# Autodesk Inventor assembly: Laufkatze_Baugruppe_neu
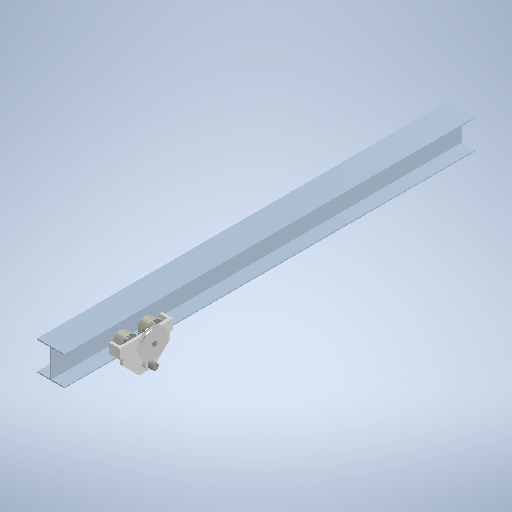
[picture p0: Inventor's stored thumbnail of the model, 512x512]
Saved by Autodesk Inventor 2025.2 (Build 292293000, 293)
## iProperties
Created: 2025-02-05
Part Number: Laufkatze_Baugruppe_neu
Document SubType Name: Assembly
Designer: akoca
Author: akoca
## Documents named in this file (16)
- C:\Users\akoca\Documents\MCI\Semester_3\AMEII\Projekt\Laufkatze\Baugruppen\Laufkatze_Baugruppe_neu.iam
- C:\Users\akoca\Documents\MCI\Semester_3\AMEII\Projekt\Laufkatze\Einzelbauteile\Stahlträger.ipt
- C:\Users\akoca\Documents\MCI\Semester_3\AMEII\Projekt\Laufkatze\Einzelbauteile\Zahnrad_für_Kettenzug.ipt
- C:\Users\akoca\Documents\MCI\Semester_3\AMEII\Projekt\Laufkatze\Einzelbauteile\Zahnrad_bei_Laufrad.ipt
- C:\Users\akoca\Documents\MCI\Semester_3\AMEII\Projekt\Laufkatze\Einzelbauteile\Laufrad.ipt
- C:\Users\akoca\Documents\MCI\Semester_3\AMEII\Projekt\Laufkatze\Einzelbauteile\Welle_für_Kettenzug.ipt
- C:\Users\akoca\Documents\MCI\Semester_3\AMEII\Projekt\Laufkatze\Einzelbauteile\Führungsplatte_rechts.ipt
- C:\Users\akoca\Documents\MCI\Semester_3\AMEII\Projekt\Laufkatze\Baugruppen\Laufkatze_Baugruppe\Konstruktions-Assistent\Lager4.iam
- C:\Users\akoca\Documents\MCI\Semester_3\AMEII\Projekt\Laufkatze\Einzelbauteile\Zugscheibe_für_Kette.ipt
- C:\Users\akoca\Documents\MCI\Semester_3\AMEII\Projekt\Laufkatze\Einzelbauteile\Führungsplatte_links.ipt
- C:\Users\akoca\Documents\MCI\Semester_3\AMEII\Projekt\Laufkatze\Einzelbauteile\Schraubbolzen.ipt
- C:\Users\akoca\Documents\MCI\Semester_3\AMEII\Projekt\Laufkatze\Baugruppen\Laufkatze_Baugruppe\Konstruktions-Assistent\Lager1.iam
- C:\Users\akoca\Documents\MCI\Semester_3\AMEII\Projekt\Laufkatze\Normteile\de-DE\DIN EN ISO 7093-2\DIN EN ISO 7093-2 - 14.ipt
- C:\Users\akoca\Documents\MCI\Semester_3\AMEII\Projekt\Laufkatze\Normteile\de-DE\ISO 8676(1)\ISO 8676 - M12 x 1,25 x 30DIN EN.ipt
- C:\Users\akoca\Documents\MCI\Semester_3\AMEII\Projekt\Laufkatze\Normteile\de-DE\DIN EN ISO 7093-2\DIN EN ISO 7093-2 - 12.ipt
- C:\Users\akoca\Documents\MCI\Semester_3\AMEII\Projekt\Laufkatze\Skelett_Laufkatze.ipt
## Components (29 placed, 13 different names)
1. DIN EN 28676 M12 x 1,25 x 30:6 — Drehbar:21
2. DIN EN ISO 7093-2 12:1 — Starr:11, Drehbar:21
3. DIN EN 28676 M12 x 1,25 x 30:5 — Starr:10
4. DIN EN 28676 M12 x 1,25 x 30:4 — Drehbar:19
5. DIN EN ISO 7093-2 14:4 — Starr:8, Drehbar:19
6. DIN EN 28676 M12 x 1,25 x 30:3 — Drehbar:20
7. DIN EN ISO 7093-2 14:3 — Starr:9, Drehbar:20
8. DIN EN 28676 M12 x 1,25 x 30:2 — Drehbar:18
9. DIN EN ISO 7093-2 14:2 — Starr:6, Drehbar:18
10. DIN EN ISO 7093-2 14:1 — Starr:7, Starr:10
11. Lager:6 [sub-assembly] — Drehbar:17
12. Lager:5 [sub-assembly] — Drehbar:16
13. Lager:4 [sub-assembly] — Drehbar:15
14. Lager:3 [sub-assembly] — Drehbar:14
15. Lager:2 [sub-assembly] — Starr:5
16. Lager:1 [sub-assembly] — Starr:4
17. Schraubbolzen:1 — Passend:7, Passend:8, Fluchtend:3
18. Laufrad:4 — Drehbar:12, Tangential:6, Drehbar:14
19. Laufrad:3 — Drehbar:13, Tangential:5, Passend:9, Drehbar:15
20. Führungsplatte_links:1 — Drehbar:12, Drehbar:13, Passend:8, Starr:6, Starr:7
21. Zugscheibe_für_Kette:1 — Drehbar:9, Drehung:3
22. Führungsplatte_rechts:1 — Drehbar:8, Drehbar:7, Passend:7, Starr:8, Starr:9, Fluchtend:4
23. Welle_für_Kettenzug:1 — Starr:4, Starr:5, Zahnrad-Bewegung, Drehbar:9, Starr:11
24. Laufrad:2 — Passend:2, Tangential:3, Starr:2, Passend:6, Drehbar:16
25. Laufrad:1 — Passend:4, Tangential:4, Starr:1, Passend:5, Drehung/Translation:1, Drehbar:17
26. Zahnrad_bei_Laufrad:2 — Fluchtend:2, Tangential:1, Passend:4, Starr:1, Drehbar:8, Drehung:2
27. Zahnrad_bei_Laufrad:1 — Fluchtend:1, Tangential:2, Passend:2, Starr:2, Drehbar:7, Drehung:1
28. Zahnrad_für_Kettenzug:1 — Fluchtend:1, Fluchtend:2, Tangential:1, Tangential:2, Drehung:1, Drehung:2, Zahnrad-Bewegung, Drehung:3
29. Stahlträger:1 — Tangential:3, Tangential:4, Passend:5, Passend:6, Drehung/Translation:1, Tangential:5, Tangential:6, Passend:9, Fluchtend:3, Fluchtend:4
## Relationships (49: RevoluteJoint 14, Mate 11, WeldJoint 10, Tangent 6, Flush 4, RelateRotation 3, RelateRotateTranslate 1)
- Fluchtend:1 [Flush]: Zahnrad_bei_Laufrad:1 ↔ Zahnrad_für_Kettenzug:1
- Fluchtend:2 [Flush]: Zahnrad_bei_Laufrad:2 ↔ Zahnrad_für_Kettenzug:1
- Tangential:1: Zahnrad_bei_Laufrad:2 ↔ Zahnrad_für_Kettenzug:1
- Tangential:2: Zahnrad_bei_Laufrad:1 ↔ Zahnrad_für_Kettenzug:1
- Passend:2 [Mate]: Laufrad:2 ↔ Zahnrad_bei_Laufrad:1
- Passend:4 [Mate]: Laufrad:1 ↔ Zahnrad_bei_Laufrad:2
- Tangential:3: Laufrad:2 ↔ Stahlträger:1
- Tangential:4: Laufrad:1 ↔ Stahlträger:1
- Starr:1 [WeldJoint]: Laufrad:1 ↔ Zahnrad_bei_Laufrad:2
- Starr:2 [WeldJoint]: Laufrad:2 ↔ Zahnrad_bei_Laufrad:1
- Drehbar:8 [RevoluteJoint] (2 mm): Führungsplatte_rechts:1 ↔ Zahnrad_bei_Laufrad:2
- Drehbar:7 [RevoluteJoint] (2 mm): Führungsplatte_rechts:1 ↔ Zahnrad_bei_Laufrad:1
- Passend:5 [Mate]: Laufrad:1 ↔ Stahlträger:1
- Passend:6 [Mate]: Laufrad:2 ↔ Stahlträger:1
- Drehung:1 [RelateRotation] (0.6 ul): Zahnrad_bei_Laufrad:1 ↔ Zahnrad_für_Kettenzug:1
- Drehung:2 [RelateRotation] (0.6 ul): Zahnrad_bei_Laufrad:2 ↔ Zahnrad_für_Kettenzug:1
- Starr:4 [WeldJoint]: Lager:1 ↔ Welle_für_Kettenzug:1
- Starr:5 [WeldJoint]: Lager:2 ↔ Welle_für_Kettenzug:1
- Zahnrad-Bewegung [RevoluteJoint]: Welle_für_Kettenzug:1 ↔ Zahnrad_für_Kettenzug:1
- Drehbar:9 [RevoluteJoint]: Zugscheibe_für_Kette:1 ↔ Welle_für_Kettenzug:1
- Drehung:3 [RelateRotation] (1 ul): Zugscheibe_für_Kette:1 ↔ Zahnrad_für_Kettenzug:1
- Drehung/Translation:1 [RelateRotateTranslate] (339.292 mm): Laufrad:1 ↔ Stahlträger:1
- Drehbar:12 [RevoluteJoint] (2 mm): Laufrad:4 ↔ Führungsplatte_links:1
- Drehbar:13 [RevoluteJoint]: Laufrad:3 ↔ Führungsplatte_links:1
- Passend:7 [Mate]: Schraubbolzen:1 ↔ Führungsplatte_rechts:1
- Passend:8 [Mate]: Schraubbolzen:1 ↔ Führungsplatte_links:1
- Tangential:5: Laufrad:3 ↔ Stahlträger:1
- Tangential:6: Laufrad:4 ↔ Stahlträger:1
- Passend:9 [Mate]: Laufrad:3 ↔ Stahlträger:1
- Fluchtend:3 [Flush]: Schraubbolzen:1 ↔ Stahlträger:1
- Drehbar:14 [RevoluteJoint]: Lager:3 ↔ Laufrad:4
- Drehbar:15 [RevoluteJoint]: Lager:4 ↔ Laufrad:3
- Drehbar:16 [RevoluteJoint]: Lager:5 ↔ Laufrad:2
- Drehbar:17 [RevoluteJoint]: Lager:6 ↔ Laufrad:1
- [Mate]: DIN EN 28676 M12 x 1,25 x 30:2 ↔ DIN EN ISO 7093-2 14:2
- [Mate]: DIN EN 28676 M12 x 1,25 x 30:3 ↔ DIN EN ISO 7093-2 14:3
- [Mate]: DIN EN 28676 M12 x 1,25 x 30:4 ↔ DIN EN ISO 7093-2 14:4
- Starr:6 [WeldJoint]: DIN EN ISO 7093-2 14:2 ↔ Führungsplatte_links:1
- Drehbar:18 [RevoluteJoint]: DIN EN 28676 M12 x 1,25 x 30:2 ↔ DIN EN ISO 7093-2 14:2
- Starr:7 [WeldJoint]: DIN EN ISO 7093-2 14:1 ↔ Führungsplatte_links:1
- Starr:8 [WeldJoint]: DIN EN ISO 7093-2 14:4 ↔ Führungsplatte_rechts:1
- Starr:9 [WeldJoint]: DIN EN ISO 7093-2 14:3 ↔ Führungsplatte_rechts:1
- Drehbar:19 [RevoluteJoint]: DIN EN 28676 M12 x 1,25 x 30:4 ↔ DIN EN ISO 7093-2 14:4
- Drehbar:20 [RevoluteJoint]: DIN EN 28676 M12 x 1,25 x 30:3 ↔ DIN EN ISO 7093-2 14:3
- Starr:10 [WeldJoint]: DIN EN 28676 M12 x 1,25 x 30:5 ↔ DIN EN ISO 7093-2 14:1
- [Mate]: DIN EN 28676 M12 x 1,25 x 30:6 ↔ DIN EN ISO 7093-2 12:1
- Starr:11 [WeldJoint]: DIN EN ISO 7093-2 12:1 ↔ Welle_für_Kettenzug:1
- Drehbar:21 [RevoluteJoint]: DIN EN 28676 M12 x 1,25 x 30:6 ↔ DIN EN ISO 7093-2 12:1
- Fluchtend:4 [Flush]: Führungsplatte_rechts:1 ↔ Stahlträger:1
## Named parameters: d90_d55 = 0 mm, d91_d55 = 0 mm, d92_d55 = 0 mm, d104_d63 = 0 mm, Traeger_laenge_l = 3000 mm, Fuehrungplatte_laenge = 348 mm, Fuehrungsplatte_breite = 20 mm
